# Autodesk Inventor assembly: Tractive Light Assembly
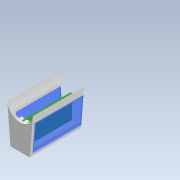
[picture p0: Inventor's stored thumbnail of the model, 180x180]
Saved by Autodesk Inventor 2021 (Build 250183000, 183)
## iProperties
Created: 2020-09-26
Part Number: Tractive Light Assembly
Document SubType Name: Assembly
Designer: capta
Author: capta
## Documents named in this file (4)
- C:\Users\capta\OneDrive - Lehigh University\Formula SAE\Tractive Light\Mount CAD\Tractive Light Assembly.iam
- C:\Users\capta\OneDrive - Lehigh University\Formula SAE\Tractive Light\Mount CAD\Tractive Light Mount.ipt
- C:\Users\capta\OneDrive - Lehigh University\Formula SAE\Tractive Light\Mount CAD\acrylic1.ipt
- C:\Users\capta\OneDrive - Lehigh University\Formula SAE\Tractive Light\Mount CAD\pcd stand in.ipt
## Components (4 placed, 3 different names)
1. Tractive Light Mount:1 — Mate:1, Mate:2, Mate:3, Mate:4, Mate:5, Mate:6, Mate:8, Mate:9
2. acrylic1:1 — Mate:1, Mate:2, Mate:3
3. acrylic1:2 — Mate:4, Mate:5, Mate:6
4. pcd stand in:1 — Mate:8, Flush:1, Flush:3
## Relationships (11: Mate 8, Flush 3)
- Mate:1: Tractive Light Mount:1 ↔ acrylic1:1
- Mate:2: Tractive Light Mount:1 ↔ acrylic1:1
- Mate:3: Tractive Light Mount:1 ↔ acrylic1:1
- Mate:4: Tractive Light Mount:1 ↔ acrylic1:2
- Mate:5: Tractive Light Mount:1 ↔ acrylic1:2
- Mate:6: Tractive Light Mount:1 ↔ acrylic1:2
- Mate:8: Tractive Light Mount:1 ↔ pcd stand in:1
- Flush:1 (-54.229 mm): pcd stand in:1
- Flush:2
- Flush:3 (-0.8128 mm): pcd stand in:1
- Mate:9: Tractive Light Mount:1
